# Autodesk Inventor assembly: z arm wall bracket
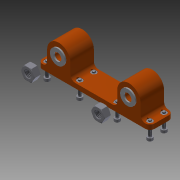
[picture p0: Inventor's stored thumbnail of the model, 180x180]
Saved by Autodesk Inventor 2014 (Build 180170000, 170)
## iProperties
Created: 2013-10-14
Part Number: z arm wall bracket
Document SubType Name: Assembly
Designer: employee
Author: employee
## Documents named in this file (6)
- \\GRISTLE\speco\GitHub\ConceptFORGE\Wally\z arm wall bracket.iam
- \\GRISTLE\speco\GitHub\ConceptFORGE\Wally\z arm wall bracket.ipt
- \\GRISTLE\speco\GitHub\ConceptFORGE\Wally\m3 nut.ipt
- \\GRISTLE\speco\GitHub\ConceptFORGE\Wally\M3x16.ipt
- \\GRISTLE\speco\GitHub\ConceptFORGE\Wally\washer.ipt
- \\GRISTLE\speco\GitHub\ConceptFORGE\Wally\M8 nut.ipt
## Components (21 placed, 5 different names)
1. z arm wall bracket:1 — Angle:1, Angle:2, Angle:3, Angle:4, Angle:5, Angle:6, Angle:7, Angle:8, Insert:1, Insert:2, Insert:3, Insert:4, Insert:5, Insert:6, Insert:7, Insert:8, Insert:9, Insert:10, Insert:11, Insert:12, Insert:13, Insert:14, Insert:15, Insert:16, Insert:17, Insert:18
2. Hex Nut Metric M3 x 0.5:1 — Angle:5, Insert:5
3. Hex Nut Metric M3 x 0.5:2 — Angle:2, Insert:2
4. Hex Nut Metric M3 x 0.5:3 — Angle:1, Insert:1
5. Hex Nut Metric M3 x 0.5:4 — Angle:3, Insert:3
6. Hex Nut Metric M3 x 0.5:5 — Angle:4, Insert:4
7. Hex Nut Metric M3 x 0.5:6 — Angle:6, Insert:8
8. Hex Nut Metric M3 x 0.5:7 — Angle:8, Insert:7
9. Hex Nut Metric M3 x 0.5:8 — Angle:7, Insert:6
10. Forged Socket Head Cap Screw - Metric M3x0.5 x 16:1 — Insert:9
11. Forged Socket Head Cap Screw - Metric M3x0.5 x 16:2 — Insert:10
12. Forged Socket Head Cap Screw - Metric M3x0.5 x 16:3 — Insert:16
13. Forged Socket Head Cap Screw - Metric M3x0.5 x 16:4 — Insert:11
14. Forged Socket Head Cap Screw - Metric M3x0.5 x 16:5 — Insert:14
15. Forged Socket Head Cap Screw - Metric M3x0.5 x 16:6 — Insert:12
16. Forged Socket Head Cap Screw - Metric M3x0.5 x 16:7 — Insert:13
17. Forged Socket Head Cap Screw - Metric M3x0.5 x 16:8 — Insert:15
18. washer:1 — Insert:18, Insert:19
19. washer:2 — Insert:17, Insert:20
20. Hex Nut Metric M8 x 1.25:1 — Insert:19
21. Hex Nut Metric M8 x 1.25:2 — Insert:20
## Relationships (28: Insert 20, Angle 8)
- Angle:1 (0 deg): z arm wall bracket:1 ↔ Hex Nut Metric M3 x 0.5:3
- Angle:2 (0 deg): z arm wall bracket:1 ↔ Hex Nut Metric M3 x 0.5:2
- Angle:3 (0 deg): z arm wall bracket:1 ↔ Hex Nut Metric M3 x 0.5:4
- Angle:4 (0 deg): z arm wall bracket:1 ↔ Hex Nut Metric M3 x 0.5:5
- Angle:5 (0 deg): z arm wall bracket:1 ↔ Hex Nut Metric M3 x 0.5:1
- Angle:6 (0 deg): z arm wall bracket:1 ↔ Hex Nut Metric M3 x 0.5:6
- Angle:7 (0 deg): z arm wall bracket:1 ↔ Hex Nut Metric M3 x 0.5:8
- Angle:8 (0 deg): z arm wall bracket:1 ↔ Hex Nut Metric M3 x 0.5:7
- Insert:1: z arm wall bracket:1 ↔ Hex Nut Metric M3 x 0.5:3
- Insert:2: z arm wall bracket:1 ↔ Hex Nut Metric M3 x 0.5:2
- Insert:3: z arm wall bracket:1 ↔ Hex Nut Metric M3 x 0.5:4
- Insert:4: z arm wall bracket:1 ↔ Hex Nut Metric M3 x 0.5:5
- Insert:5: z arm wall bracket:1 ↔ Hex Nut Metric M3 x 0.5:1
- Insert:6: z arm wall bracket:1 ↔ Hex Nut Metric M3 x 0.5:8
- Insert:7: z arm wall bracket:1 ↔ Hex Nut Metric M3 x 0.5:7
- Insert:8: z arm wall bracket:1 ↔ Hex Nut Metric M3 x 0.5:6
- Insert:9 (9.5 mm): z arm wall bracket:1 ↔ Forged Socket Head Cap Screw - Metric M3x0.5 x 16:1
- Insert:10 (9.5 mm): z arm wall bracket:1 ↔ Forged Socket Head Cap Screw - Metric M3x0.5 x 16:2
- Insert:11 (9.5 mm): z arm wall bracket:1 ↔ Forged Socket Head Cap Screw - Metric M3x0.5 x 16:4
- Insert:12 (9.5 mm): z arm wall bracket:1 ↔ Forged Socket Head Cap Screw - Metric M3x0.5 x 16:6
- Insert:13 (9.5 mm): z arm wall bracket:1 ↔ Forged Socket Head Cap Screw - Metric M3x0.5 x 16:7
- Insert:14 (9.5 mm): z arm wall bracket:1 ↔ Forged Socket Head Cap Screw - Metric M3x0.5 x 16:5
- Insert:15 (9.5 mm): z arm wall bracket:1 ↔ Forged Socket Head Cap Screw - Metric M3x0.5 x 16:8
- Insert:16 (9.5 mm): z arm wall bracket:1 ↔ Forged Socket Head Cap Screw - Metric M3x0.5 x 16:3
- Insert:17: z arm wall bracket:1 ↔ washer:2
- Insert:18: z arm wall bracket:1 ↔ washer:1
- Insert:19 (25 mm): washer:1 ↔ Hex Nut Metric M8 x 1.25:1
- Insert:20 (25 mm): washer:2 ↔ Hex Nut Metric M8 x 1.25:2
